# Autodesk Inventor assembly: Xcr
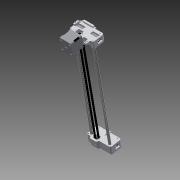
[picture p0: Inventor's stored thumbnail of the model, 180x180]
Saved by Autodesk Inventor 2013 (Build 170138000, 138)
## iProperties
Created: 2015-01-14
Part Number: Xcr
Document SubType Name: Assembly
Designer: dzban
Author: dzban
## Documents named in this file (5)
- D:\PIRX\Artisan\OPENSOURCE\XCars\Xcr.iam
- D:\PIRX\Artisan\OPENSOURCE\XCars\XcrRight.iam
- D:\PIRX\Artisan\OPENSOURCE\XCars\XcrLeft.iam
- D:\PIRX\Artisan\OPENSOURCE\XCars\Yshaft.ipt
- D:\PIRX\Artisan\OPENSOURCE\StockComponents\gt2Belt760.ipt
## Components (5 placed, 4 different names)
1. XcrRight:1 [sub-assembly] — Insert:1, Insert:2, Insert:5, Angle:1
2. XcrLeft:1 [sub-assembly] — Insert:3, Insert:4
3. Yshaft:1 — Insert:2, Insert:3
4. Yshaft:2 — Insert:1, Insert:4
5. gt2Belt760:1 — Insert:5, Angle:1
## Relationships (6: Insert 5, Angle 1)
- Insert:1 (-18 mm): XcrRight:1 ↔ Yshaft:2
- Insert:2 (-18 mm): XcrRight:1 ↔ Yshaft:1
- Insert:3 (-18 mm): XcrLeft:1 ↔ Yshaft:1
- Insert:4 (-18 mm): XcrLeft:1 ↔ Yshaft:2
- Insert:5: XcrRight:1 ↔ gt2Belt760:1
- Angle:1 (0 deg): XcrRight:1 ↔ gt2Belt760:1
